# Autodesk Inventor assembly: printplaat
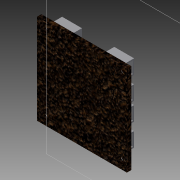
[picture p0: Inventor's stored thumbnail of the model, 180x180]
Saved by Autodesk Inventor 2015 (Build 190159000, 159)
## iProperties
Created: 2015-12-04
Part Number: printplaat
Document SubType Name: Assembly
Designer: david
Author: david
## Documents named in this file (4)
- Z:\gip\Inventor\generatie 7\Frame\Electronica\printplaat\printplaat.iam
- Z:\gip\Inventor\generatie 7\Frame\Electronica\printplaat\print.ipt
- Z:\gip\Inventor\generatie 7\Frame\Electronica\printplaat\netwerk.ipt
- Z:\gip\Inventor\generatie 7\Frame\Electronica\printplaat\blokken.iam
## Components (10 placed, 3 different names)
1. print:1 — Mate:1, Flush:1, Flush:2, Mate:2, Flush:3, Flush:4, Mate:3, Flush:5, Flush:6
2. blokken:1 [sub-assembly] — Mate:3, Flush:5, Flush:6
3. netwerk:2 — Mate:1, Flush:1, Flush:2
4. netwerk:3
5. netwerk:4
6. netwerk:5
7. netwerk:7 — Mate:2, Flush:3, Flush:4
8. netwerk:8
9. netwerk:9
10. netwerk:10
## Component patterns: (2 elements), (2 elements), (2 elements, first: netwerk:2), Component Pattern 1:2 (2 elements), (2 elements, first: netwerk:7), Component Pattern 3:2 (2 elements)
## Relationships (9: Flush 6, Mate 3)
- Mate:1: print:1 ↔ netwerk:2
- Flush:1 (10 mm): print:1 ↔ netwerk:2
- Flush:2 (10 mm): print:1 ↔ netwerk:2
- Mate:2: print:1 ↔ netwerk:7
- Flush:3 (10 mm): print:1 ↔ netwerk:7
- Flush:4 (10 mm): print:1 ↔ netwerk:7
- Mate:3: print:1 ↔ blokken:1
- Flush:5 (40 mm): print:1 ↔ blokken:1
- Flush:6 (20 mm): print:1 ↔ blokken:1
